# Autodesk Inventor assembly: 5 Barras Version 0
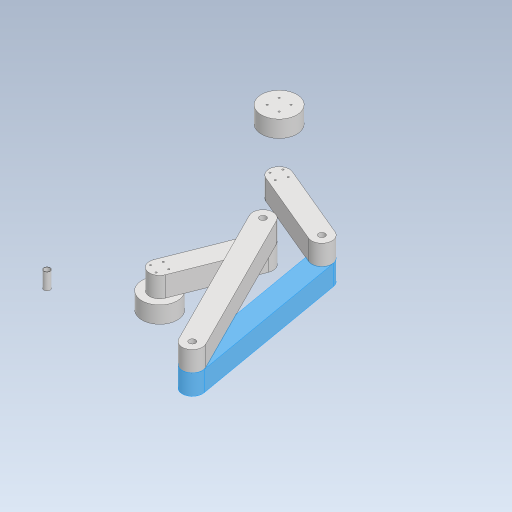
[picture p0: Inventor's stored thumbnail of the model, 512x512]
Saved by Autodesk Inventor 2024.2 (Build 282272000, 272)
## iProperties
Created: 2025-02-06
Part Number: 5 Barras Version 0
Document SubType Name: Assembly
Designer: jp.reyesf
Author: jp.reyesf
## Documents named in this file (7)
- C:\Users\jp.reyesf\Desktop\Master-Thesis\five_bar\assets\CAD\test\5 Barras Version 0.iam
- C:\Users\jp.reyesf\Desktop\Master-Thesis\five_bar\assets\CAD\test\Solid6.ipt
- C:\Users\jp.reyesf\Desktop\Master-Thesis\five_bar\assets\CAD\test\Solid7.ipt
- C:\Users\jp.reyesf\Desktop\Master-Thesis\five_bar\assets\CAD\test\Solid8.ipt
- C:\Users\jp.reyesf\Desktop\Master-Thesis\five_bar\assets\CAD\test\Solid9.ipt
- C:\Users\jp.reyesf\Desktop\Master-Thesis\five_bar\assets\CAD\test\Solid13.ipt
- C:\Users\jp.reyesf\Desktop\Master-Thesis\five_bar\assets\CAD\test\Solid14.ipt
## Components (6 placed, 6 different names)
1. Solid6:1 — Mate:1, Mate:2, Mate:3, Mate:4
2. Solid7:1 — Mate:3, Mate:4, Mate:5, Mate:6
3. Solid8:1 — Mate:5, Mate:6, Mate:7, Mate:8
4. Solid9:1 — Mate:7, Mate:8, Mate:9
5. Solid13:1
6. Solid14:1 — Mate:1, Mate:2, Mate:9
## Relationships (9: Mate 9)
- Mate:1: Solid6:1 ↔ Solid14:1
- Mate:2: Solid6:1 ↔ Solid14:1
- Mate:3: Solid6:1 ↔ Solid7:1
- Mate:4: Solid6:1 ↔ Solid7:1
- Mate:5: Solid7:1 ↔ Solid8:1
- Mate:6: Solid7:1 ↔ Solid8:1
- Mate:7: Solid8:1 ↔ Solid9:1
- Mate:8: Solid8:1 ↔ Solid9:1
- Mate:9: Solid9:1 ↔ Solid14:1
